# Autodesk Inventor assembly: Token design 2
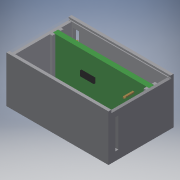
[picture p0: Inventor's stored thumbnail of the model, 180x180]
Saved by Autodesk Inventor 2018.3 (Build 223284000, 284)
## iProperties
Created: 2020-11-10
Part Number: Token design 2
Document SubType Name: Assembly
Designer: daanv
Author: daanv
## Documents named in this file (6)
- C:\Users\daanv\OneDrive\Documenten\Life\Avans Project RED\Token\Design 2\Token design 2.iam
- C:\Users\daanv\OneDrive\Documenten\Life\Avans Project RED\Token\Design 2\Onderkant.ipt
- C:\Users\daanv\OneDrive\Documenten\Life\Avans Project RED\Token\Design 2\Zijkant 1.ipt
- C:\Users\daanv\OneDrive\Documenten\Life\Avans Project RED\Token\Design 2\Zijkant 2.ipt
- C:\Users\daanv\OneDrive\Documenten\Life\Avans Project RED\Token\Design 2\Zijkant 3.ipt
- C:\Users\daanv\OneDrive\Documenten\Life\Avans Project RED\Token\Design 2\Zijkant 4.ipt
## Components (5 placed, 5 different names)
1. Onderkant:1 — Mate:2, Mate:3, Mate:4, Mate:5, Mate:9, Mate:10
2. Zijkant 1:1 — Mate:2, Mate:3, Mate:11, Mate:21
3. Zijkant 2:1 — Mate:4, Mate:5
4. Zijkant 3:1 — Mate:10, Mate:11
5. Zijkant 4:1 — Mate:9, Mate:21
## Relationships (8: Mate 8)
- Mate:2: Onderkant:1 ↔ Zijkant 1:1
- Mate:3: Onderkant:1 ↔ Zijkant 1:1
- Mate:4: Onderkant:1 ↔ Zijkant 2:1
- Mate:5: Onderkant:1 ↔ Zijkant 2:1
- Mate:9: Onderkant:1 ↔ Zijkant 4:1
- Mate:10: Onderkant:1 ↔ Zijkant 3:1
- Mate:11: Zijkant 1:1 ↔ Zijkant 3:1
- Mate:21: Zijkant 1:1 ↔ Zijkant 4:1
